# Autodesk Inventor assembly: Drawback 1
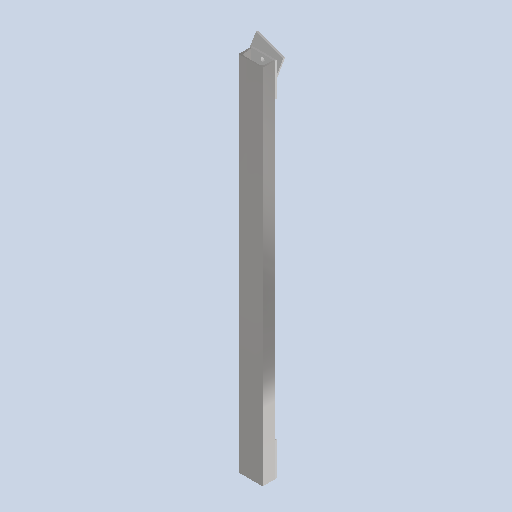
[picture p0: Inventor's stored thumbnail of the model, 512x512]
Saved by Autodesk Inventor 2025 (Build 290162010, 162A)
## iProperties
Created: 2024-07-04
Part Number: Drawback 1
Document SubType Name: Assembly
Designer: pokla
Stock Number: Оттяжка 1
Author: pokla
## Documents named in this file (4)
- C:\Users\pokla\Documents\Inventor\Goat\Оттяжки.iam
- C:\Users\pokla\Documents\Inventor\Goat\Сrane plate 5.1.ipt
- C:\Users\pokla\Documents\Inventor\Goat\Сhannel.ipt
- C:\Users\pokla\Documents\Inventor\Goat\Сrane plate 5.ipt
## Components (4 placed, 3 different names)
1. Сrane plate 5.1.ipt:1
2. Сhannel.ipt:1
3. Сrane plate 5.1.ipt:2
4. Сrane plate 5.ipt:2
## Relationships (8: Flush 4, Mate 3, RevoluteJoint 1)
- [Flush]: Сrane plate 5.1.ipt:1 ↔ Сhannel.ipt:1
- [Flush]: Сrane plate 5.1.ipt:1 ↔ Сhannel.ipt:1
- [Mate]: Сrane plate 5.1.ipt:1 ↔ Сhannel.ipt:1
- [Flush]: Сhannel.ipt:1 ↔ Сrane plate 5.1.ipt:2
- [Flush]: Сhannel.ipt:1 ↔ Сrane plate 5.1.ipt:2
- [Mate]: Сhannel.ipt:1 ↔ Сrane plate 5.1.ipt:2
- [RevoluteJoint]: Сrane plate 5.1.ipt:2 ↔ Сrane plate 5.ipt:2
- [Mate]: Сrane plate 5.1.ipt:2 ↔ Сrane plate 5.ipt:2
## Named parameters: d52_d65 = 0 mm, d53_d66 = 0 mm, d54_d67 = 0 mm, d55_d68 = 0 mm
